# Autodesk Inventor assembly: MEC-ASM-1000-F450_Frame
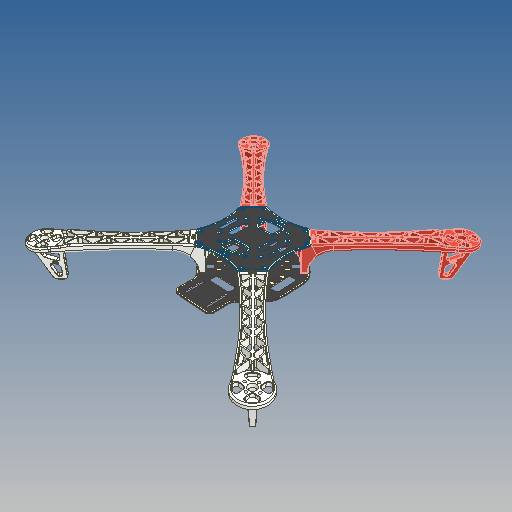
[picture p0: Inventor's stored thumbnail of the model, 512x512]
Saved by Autodesk Inventor 2026 (Build 300175000, 175)
## iProperties
Created: 2026-07-22
Part Number: MEC-ASM-1000-F450_Frame
Document SubType Name: Assembly
Designer: Pacman Ng
Mass: 303.023 g
Surface Area: 1534.12 cm^2
Volume: 190.337 cm^3
Density: 1.59204 g/cm^3
Author: Pacman Ng
## Documents named in this file (5)
- D:\OneDrive_MSFT\Work\Drone Research\3d_models\Full_body\MEC-ASM-1000-F450_Frame.iam
- D:\OneDrive_MSFT\Work\Drone Research\3d_models\Full_body\MEC-PRT-1001-Base_Top.ipt
- D:\OneDrive_MSFT\Work\Drone Research\3d_models\Full_body\MEC-PRT-1002-Base_Bottom.ipt
- D:\OneDrive_MSFT\Work\Drone Research\3d_models\Full_body\MEC-PRT-1003-Arm_White.ipt
- D:\OneDrive_MSFT\Work\Drone Research\3d_models\Full_body\MEC-PRT-1004-Arm_Red.ipt
## Components (6 placed, 4 different names)
1. MEC-PRT-1001-Base_Top:1 — Flush:1, Flush:2, Flush:3, Mate:1, Mate:2, Mate:3, Mate:4, Mate:5, Mate:6, Mate:7, Mate:8, Mate:9, Mate:10, Mate:11, Mate:12
2. MEC-PRT-1002-Base_Bottom:1 — Mate:13, Mate:14, Mate:15
3. MEC-PRT-1003-Arm_White:1 — Mate:2, Mate:3, Mate:6
4. MEC-PRT-1003-Arm_White:2 — Mate:1, Mate:4, Mate:5, Mate:15
5. MEC-PRT-1004-Arm_Red:1 — Mate:8, Mate:11, Mate:12, Mate:14
6. MEC-PRT-1004-Arm_Red:2 — Mate:7, Mate:9, Mate:10, Mate:13
## Relationships (18: Mate 15, Flush 3)
- Flush:1: MEC-PRT-1001-Base_Top:1
- Flush:2 (-18 mm): MEC-PRT-1001-Base_Top:1
- Flush:3 (-18 mm): MEC-PRT-1001-Base_Top:1
- Mate:1: MEC-PRT-1001-Base_Top:1 ↔ MEC-PRT-1003-Arm_White:2
- Mate:2: MEC-PRT-1001-Base_Top:1 ↔ MEC-PRT-1003-Arm_White:1
- Mate:3: MEC-PRT-1001-Base_Top:1 ↔ MEC-PRT-1003-Arm_White:1
- Mate:4: MEC-PRT-1001-Base_Top:1 ↔ MEC-PRT-1003-Arm_White:2
- Mate:5: MEC-PRT-1001-Base_Top:1 ↔ MEC-PRT-1003-Arm_White:2
- Mate:6: MEC-PRT-1001-Base_Top:1 ↔ MEC-PRT-1003-Arm_White:1
- Mate:7: MEC-PRT-1001-Base_Top:1 ↔ MEC-PRT-1004-Arm_Red:2
- Mate:8: MEC-PRT-1001-Base_Top:1 ↔ MEC-PRT-1004-Arm_Red:1
- Mate:9: MEC-PRT-1001-Base_Top:1 ↔ MEC-PRT-1004-Arm_Red:2
- Mate:10: MEC-PRT-1001-Base_Top:1 ↔ MEC-PRT-1004-Arm_Red:2
- Mate:11: MEC-PRT-1001-Base_Top:1 ↔ MEC-PRT-1004-Arm_Red:1
- Mate:12: MEC-PRT-1001-Base_Top:1 ↔ MEC-PRT-1004-Arm_Red:1
- Mate:13: MEC-PRT-1002-Base_Bottom:1 ↔ MEC-PRT-1004-Arm_Red:2
- Mate:14: MEC-PRT-1002-Base_Bottom:1 ↔ MEC-PRT-1004-Arm_Red:1
- Mate:15: MEC-PRT-1002-Base_Bottom:1 ↔ MEC-PRT-1003-Arm_White:2
